# Autodesk Inventor assembly: LIBS分光系
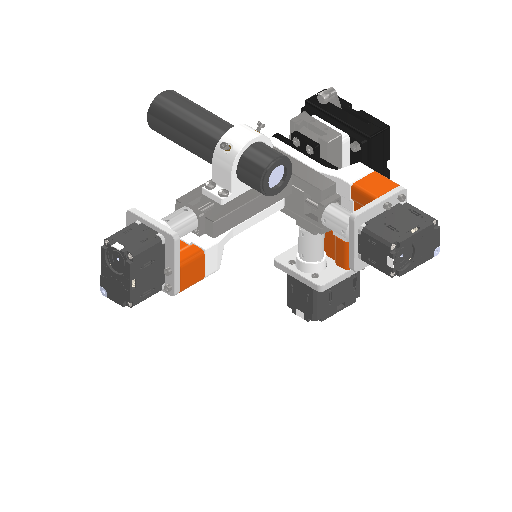
[picture p0: Inventor's stored thumbnail of the model, 512x512]
Saved by Autodesk Inventor 2026.2 (Build 302298000, 298)
## iProperties
Created: 2025-07-15
Part Number: LIBS分光系
Document SubType Name: Assembly
Designer: jin20
Author: jin20
## Documents named in this file (4)
- D:\repos\PIHTI\SpectroscopySystem_Hayashi\LIBS分光系.iam
- D:\repos\PIHTI\SpectroscopySystem_Hayashi\Stage\マグネットベース.ipt
- D:\repos\PIHTI\SpectroscopySystem_Hayashi\Optics\チューブレンズ_縮尺変更.ipt
- D:\repos\PIHTI\LIBS\XL430-bracket.iam
## Components (3 placed, 3 different names)
1. マグネットベース:1 — メイト:1, メイト:2, メイト:3
2. チューブレンズ_縮尺変更:1 — メイト:4
3. XL430-bracket:1 [sub-assembly] — メイト:1, メイト:2, メイト:3, メイト:4
## Relationships (4: Mate 4)
- メイト:1 [Mate]: マグネットベース:1 ↔ XL430-bracket:1
- メイト:2 [Mate]: マグネットベース:1 ↔ XL430-bracket:1
- メイト:3 [Mate] (0.424 mm): マグネットベース:1 ↔ XL430-bracket:1
- メイト:4 [Mate]: チューブレンズ_縮尺変更:1 ↔ XL430-bracket:1
